# Autodesk Inventor assembly: 276-2177 + 276-1321
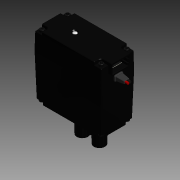
[picture p0: Inventor's stored thumbnail of the model, 180x180]
Saved by Autodesk Inventor 2016 (Build 200138000, 138)
## iProperties
Category: Motion & Sensors
Company: Super Sonic Sparks, Team 24
Part Number: 276-2177 + 276-1321
Document SubType Name: Assembly
Designer: Jordan Kiesel
Mass: 87.09 g
Surface Area: 402.615 cm^2
Volume: 32.8211 cm^3
Catalog Web Link: vexrobotics.com/276-2177.html & vexrobotics.com/276-1321.html
Description: 60% more output power than the standard motor, with an added quadrature encoder.
Vendor: VEX Robotics, Inc.
Density: 2.65348 g/cm^3
Translation Standard: STEP AP203
FileName: 2-Wire Motor 393-Integrated Encoder Module.iam
PreProcessor: SolidWorks 2009
PostProcessor: Build: 239, Release: 2011 RTM - Date: Wed 02/17/2010
Sent Units: inch
Uncertainty: 1e-05
Author: Jordan Kiesel
Title: 2-Wire Motor 393-Integrated Encoder Module
Comments: The 2 Wire Motor 393 provides 60% more output power than the standard motor, which allows for more powerful mechanisms and drive bases. ▷ Strong, steel internal gears. ▷ No clutches needed. ▷ Can be configured into a "high speed" version. ▷ Has 60% more torque than the 3-wire VEX Motor. The 2-Wire Motor 393 does not have an internal motor controller. The motor connects directly to 2-Wire Motor Ports (Ports 1 & 10 on the Cortex Microcontroller). For 3-Wire Motor Ports (Ports 2-9 on the Cortex), a Motor Controller 29 must be used in between the Microcontroller and the motor. The Integrated Encoder Module replaces the plastic cap on the back of a VEX 2-Wire Motor 393 with a quadrature encoder. Install this product and connect it to your Cortex Microcontroller via I2C to receive direct feedback from the motor. This encoder provides information on how fast the motor is going, how far it has traveled, and what direction it is moving. ▷ Increased feedback from your motors allows for more control. ▷ Communicates via I2C via included 4-wire Cable. ▷ Not compatible with the PIC Microcontroller. ▷ Programming Required! Consult your software provider for details.
## Documents named in this file (21)
- C:\Users\Jordan\Documents\Robotics\CAD\2015 BNS CAD Library (beta)\Motion\Motors\2-Wire Motor 393, Integrated Encoder Module.iam
- C:\Users\Jordan\Documents\Robotics\CAD\2015 BNS CAD Library (beta)\Motion\Motors\Reference Parts\2-Wire Motors\0.589'' Screw.ipt
- C:\Users\Jordan\Documents\Robotics\CAD\2015 BNS CAD Library (beta)\Motion\Motors\Reference Parts\2-Wire Motor 393\0.197'' Screw.ipt
- C:\Users\Jordan\Documents\Robotics\CAD\2015 BNS CAD Library (beta)\Motion\Motors\Reference Parts\2-Wire Motor 393\Bottom Housing.ipt
- C:\Users\Jordan\Documents\Robotics\CAD\2015 BNS CAD Library (beta)\Motion\Motors\Reference Parts\2-Wire Motor 393\32-tooth Output Gear (High Torque).ipt
- C:\Users\Jordan\Documents\Robotics\CAD\2015 BNS CAD Library (beta)\Motion\Motors\Reference Parts\2-Wire Motor 393\0.819'' Shaft.ipt
- C:\Users\Jordan\Documents\Robotics\CAD\2015 BNS CAD Library (beta)\Motion\Motors\Reference Parts\2-Wire Motor 393\Bearing.ipt
- C:\Users\Jordan\Documents\Robotics\CAD\2015 BNS CAD Library (beta)\Motion\Motors\Reference Parts\Motors\2-Wire Cable Support.ipt
- C:\Users\Jordan\Documents\Robotics\CAD\2015 BNS CAD Library (beta)\Motion\Motors\Reference Parts\2-Wire Motor 393\Internal Motor Carrier.ipt
- C:\Users\Jordan\Documents\Robotics\CAD\2015 BNS CAD Library (beta)\Motion\Motors\Reference Parts\2-Wire Motors\6-32 Screw Insert Nut.ipt
- C:\Users\Jordan\Documents\Robotics\CAD\2015 BNS CAD Library (beta)\Motion\Motors\Reference Parts\2-Wire Motors\2-Wire Motor Cable, Cut.ipt
- C:\Users\Jordan\Documents\Robotics\CAD\2015 BNS CAD Library (beta)\Motion\Motors\Reference Parts\2-Wire Motor 393\12-tooth Input Gear.ipt
- C:\Users\Jordan\Documents\Robotics\CAD\2015 BNS CAD Library (beta)\Motion\Motors\Reference Parts\2-Wire Motor 393\Internal Motor.ipt
- C:\Users\Jordan\Documents\Robotics\CAD\2015 BNS CAD Library (beta)\Motion\Motors\Reference Parts\2-Wire Motor 393\12-49-tooth Compound Gear.ipt
- C:\Users\Jordan\Documents\Robotics\CAD\2015 BNS CAD Library (beta)\Motion\Motors\Reference Parts\2-Wire Motor 393\1.083'' Shaft.ipt
- C:\Users\Jordan\Documents\Robotics\CAD\2015 BNS CAD Library (beta)\Motion\Motors\Reference Parts\2-Wire Motor 393\0.583'' Shaft.ipt
- C:\Users\Jordan\Documents\Robotics\CAD\2015 BNS CAD Library (beta)\Motion\Motors\Reference Parts\2-Wire Motor 393\10-33-tooth Compound Gear (High Torque).ipt
- C:\Users\Jordan\Documents\Robotics\CAD\2015 BNS CAD Library (beta)\Motion\Motors\Reference Parts\2-Wire Motor 393\Large Bearing.ipt
- C:\Users\Jordan\Documents\Robotics\CAD\2015 BNS CAD Library (beta)\Motion\Motors\Reference Parts\2-Wire Motor 393\Top Housing.ipt
- C:\Users\Jordan\Documents\Robotics\CAD\2015 BNS CAD Library (beta)\Motion\Motors\Reference Parts\2-Wire Motor 393, Integrated Encoder Module\Motor 393 Integrated Encoder Module.iam
- C:\Users\Jordan\Documents\Robotics\CAD\2015 BNS CAD Library (beta)\Motion\Motors\Reference Parts\2-Wire Motor 393, Integrated Encoder Module\11-48-tooth Compound Gear, Labeled.iam
## Components (29 placed, 20 different names)
1. 0.589'' Screw:1 — Insert:3
2. 0.589'' Screw:2 — Insert:2
3. 0.197'' Screw:1 — Insert:24
4. Bottom Housing:1 — Insert:7, Insert:8, Insert:20, Insert:21, Insert:22, Insert:23, Insert:24, Insert:25, Insert:26
5. 0.589'' Screw:3 — Insert:1
6. 32-tooth Output Gear (High Torque):1 — Insert:10, Insert:12, Rotation:1
7. 0.819'' Shaft:1 — Insert:26
8. Motor 393 Integrated Encoder Module:1 [sub-assembly] — Insert:16, Insert:17, Insert:18, Insert:19, Insert:20, Insert:21, Insert:27
9. Bearing:1 — Insert:10
10. 2-Wire Cable Support:1
11. Internal Motor Carrier:1 — Insert:9, Angle:1
12. 6-32 Screw Insert Nut:1 — Insert:5
13. 2-Wire Motor Cable, Cut:1
14. 0.589'' Screw:4 — Insert:18
15. 12-tooth Input Gear:1 — Insert:15, Rotation:4
16. 0.589'' Screw:5 — Insert:16
17. 6-32 Screw Insert Nut:2 — Insert:6
18. 0.197'' Screw:2 — Insert:25
19. Internal Motor:1 — Insert:9, Angle:1, Insert:15
20. 12-49-tooth Compound Gear:1 — Insert:27, Rotation:2, Rotation:3
21. 1.083'' Shaft:1 — Insert:14
22. 0.583'' Shaft:1 — Insert:22
23. 10-33-tooth Compound Gear (High Torque):1 — Insert:13, Rotation:1, Rotation:2
24. Large Bearing:1 — Insert:11, Insert:12
25. 0.589'' Screw:6 — Insert:17
26. Top Housing:1 — Insert:1, Insert:2, Insert:3, Insert:4, Insert:5, Insert:6, Insert:7, Insert:8, Insert:11, Insert:13, Insert:14
27. 0.589'' Screw:7 — Insert:19
28. 11-48-tooth Compound Gear, Labeled:1 [sub-assembly] — Insert:23, Rotation:3, Rotation:4
29. 0.589'' Screw:8 — Insert:4
## Relationships (32: Insert 27, RelateRotation 4, Angle 1)
- Insert:1: 0.589'' Screw:3 ↔ Top Housing:1
- Insert:2: 0.589'' Screw:2 ↔ Top Housing:1
- Insert:3: 0.589'' Screw:1 ↔ Top Housing:1
- Insert:4: Top Housing:1 ↔ 0.589'' Screw:8
- Insert:5: 6-32 Screw Insert Nut:1 ↔ Top Housing:1
- Insert:6: 6-32 Screw Insert Nut:2 ↔ Top Housing:1
- Insert:7: Bottom Housing:1 ↔ Top Housing:1
- Insert:8: Bottom Housing:1 ↔ Top Housing:1
- Insert:9: Internal Motor Carrier:1 ↔ Internal Motor:1
- Angle:1 (0 deg): Internal Motor Carrier:1 ↔ Internal Motor:1
- Insert:10: 32-tooth Output Gear (High Torque):1 ↔ Bearing:1
- Insert:11: Large Bearing:1 ↔ Top Housing:1
- Insert:12: 32-tooth Output Gear (High Torque):1 ↔ Large Bearing:1
- Insert:13: 10-33-tooth Compound Gear (High Torque):1 ↔ Top Housing:1
- Insert:14: 1.083'' Shaft:1 ↔ Top Housing:1
- Insert:15 (0.889 mm): 12-tooth Input Gear:1 ↔ Internal Motor:1
- Insert:16: Motor 393 Integrated Encoder Module:1 ↔ 0.589'' Screw:5
- Insert:17: Motor 393 Integrated Encoder Module:1 ↔ 0.589'' Screw:6
- Insert:18: Motor 393 Integrated Encoder Module:1 ↔ 0.589'' Screw:4
- Insert:19: Motor 393 Integrated Encoder Module:1 ↔ 0.589'' Screw:7
- Insert:20: Bottom Housing:1 ↔ Motor 393 Integrated Encoder Module:1
- Insert:21: Bottom Housing:1 ↔ Motor 393 Integrated Encoder Module:1
- Insert:22: Bottom Housing:1 ↔ 0.583'' Shaft:1
- Insert:23 (0.2032 mm): Bottom Housing:1 ↔ 11-48-tooth Compound Gear, Labeled:1
- Insert:24: 0.197'' Screw:1 ↔ Bottom Housing:1
- Insert:25: Bottom Housing:1 ↔ 0.197'' Screw:2
- Insert:26: Bottom Housing:1 ↔ 0.819'' Shaft:1
- Insert:27: Motor 393 Integrated Encoder Module:1 ↔ 12-49-tooth Compound Gear:1
- Rotation:1 [RelateRotation] (3.2 ul): 32-tooth Output Gear (High Torque):1 ↔ 10-33-tooth Compound Gear (High Torque):1
- Rotation:2 [RelateRotation] (2.75 ul): 12-49-tooth Compound Gear:1 ↔ 10-33-tooth Compound Gear (High Torque):1
- Rotation:3 [RelateRotation] (4.4545 ul): 12-49-tooth Compound Gear:1 ↔ 11-48-tooth Compound Gear, Labeled:1
- Rotation:4 [RelateRotation] (4 ul): 12-tooth Input Gear:1 ↔ 11-48-tooth Compound Gear, Labeled:1
